# Autodesk Inventor assembly: 草图
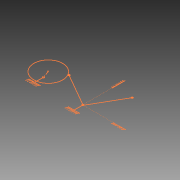
[picture p0: Inventor's stored thumbnail of the model, 180x180]
Saved by Autodesk Inventor 2011 SP1 (Build 150282100, 282)
## iProperties
Created: 2012-03-19
Part Number: 草图
Document SubType Name: Assembly
Designer: Zhensheng
Author: Zhensheng
## Documents named in this file (5)
- E:\inventor\概念设计\草图.iam
- E:\inventor\概念设计\草图.ipt
- E:\inventor\概念设计\地.ipt
- E:\inventor\概念设计\连杆.ipt
- E:\inventor\概念设计\偏心轮.ipt
## Components (4 placed, 4 different names)
1. 草图:1
2. 地:1 — 配合:1, 配合:2
3. 连杆:1 — 配合:2
4. 偏心轮:1 — 配合:1
## Relationships (5: Composite 3, Mate 2)
- [Composite]: 草图:1 ↔ 地:1
- [Composite]: 草图:1 ↔ 连杆:1
- [Composite]: 草图:1 ↔ 偏心轮:1
- 配合:1 [Mate]: 地:1 ↔ 偏心轮:1
- 配合:2 [Mate]: 地:1 ↔ 连杆:1
